# Autodesk Inventor assembly: X Axis Assembly 1.0
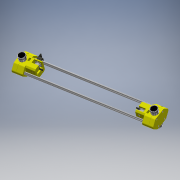
[picture p0: Inventor's stored thumbnail of the model, 180x180]
Saved by Autodesk Inventor 2016 (Build 200138000, 138)
## iProperties
Created: 2017-04-09
Part Number: X Axis Assembly 1.0
Document SubType Name: Assembly
Designer: Scott
Author: Scott
## Documents named in this file (5)
- E:\Scott Projects\3D Printing\CoreXY\X Axis Assembly 1.0.iam
- E:\Scott Projects\3D Printing\CoreXY\Y Carriage Assemby 1.0.iam
- E:\Scott Projects\3D Printing\CoreXY\Linear rail - X.ipt
- E:\Scott Projects\3D Printing\CoreXY\LM10UU.ipt
- E:\Scott Projects\3D Printing\CoreXY\Y End Stop Flag.ipt
## Components (9 placed, 4 different names)
1. Y Carriage Assemby 1.0:1 [sub-assembly] — Mate:1, Mate:2, Flush:1, Flush:2, Mate:9, Flush:4, Flush:6, Angle:1
2. Linear rail - X:1 — Mate:1, Flush:1, Mate:3, Flush:3, Mate:11
3. Linear rail - X:2 — Mate:2, Flush:2, Mate:4
4. Y Carriage Assemby 1.0:2 [sub-assembly] — Mate:3, Mate:4, Flush:3, Mate:10, Flush:5
5. LM10UU:1 — Mate:5, Mate:6, Mate:9
6. LM10UU:2 — Mate:5, Mate:6, Flush:4
7. LM10UU:3 — Mate:7, Mate:8, Mate:10
8. LM10UU:4 — Mate:7, Mate:8, Flush:5
9. Y End Stop Flag:1 — Mate:11, Flush:6, Angle:1
## Relationships (18: Mate 11, Flush 6, Angle 1)
- Mate:1: Y Carriage Assemby 1.0:1 ↔ Linear rail - X:1
- Mate:2: Y Carriage Assemby 1.0:1 ↔ Linear rail - X:2
- Flush:1: Y Carriage Assemby 1.0:1 ↔ Linear rail - X:1
- Flush:2: Y Carriage Assemby 1.0:1 ↔ Linear rail - X:2
- Mate:3: Linear rail - X:1 ↔ Y Carriage Assemby 1.0:2
- Mate:4: Linear rail - X:2 ↔ Y Carriage Assemby 1.0:2
- Flush:3: Linear rail - X:1 ↔ Y Carriage Assemby 1.0:2
- Mate:5: LM10UU:1 ↔ LM10UU:2
- Mate:6: LM10UU:1 ↔ LM10UU:2
- Mate:7: LM10UU:3 ↔ LM10UU:4
- Mate:8: LM10UU:3 ↔ LM10UU:4
- Mate:9: Y Carriage Assemby 1.0:1 ↔ LM10UU:1
- Mate:10: Y Carriage Assemby 1.0:2 ↔ LM10UU:3
- Flush:4 (-14 mm): Y Carriage Assemby 1.0:1 ↔ LM10UU:2
- Flush:5 (-14 mm): Y Carriage Assemby 1.0:2 ↔ LM10UU:4
- Mate:11: Linear rail - X:1 ↔ Y End Stop Flag:1
- Flush:6 (10 mm): Y Carriage Assemby 1.0:1 ↔ Y End Stop Flag:1
- Angle:1 (0 deg): Y Carriage Assemby 1.0:1 ↔ Y End Stop Flag:1
